# Autodesk Inventor assembly: MECANISMO DE COMPACTADO
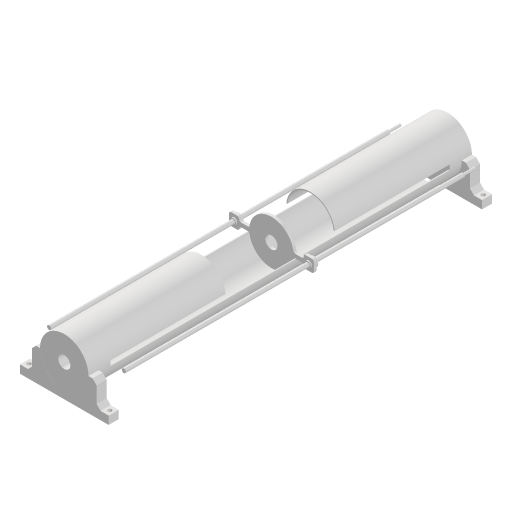
[picture p0: Inventor's stored thumbnail of the model, 512x512]
Saved by Autodesk Inventor 2024 (Build 280153000, 153)
## iProperties
Created: 2024-05-26
Part Number: MECANISMO DE COMPACTADO
Document SubType Name: Assembly
Designer: Jhuliams
Author: Jhuliams
## Documents named in this file (6)
- C:\Users\Jhuliams\Documents\GitHub\RECICLADOR_MODELO_3D\MECANISMO DE COMPACTADO\MECANISMO DE COMPACTADO.iam
- C:\Users\Jhuliams\Documents\GitHub\RECICLADOR_MODELO_3D\MECANISMO DE COMPACTADO\GUIA_DE_OBJETO.ipt
- C:\Users\Jhuliams\Documents\GitHub\RECICLADOR_MODELO_3D\MECANISMO DE COMPACTADO\TAPA QUE DESPLAZA CON TORNILLOS.ipt
- C:\Users\Jhuliams\Documents\GitHub\RECICLADOR_MODELO_3D\MECANISMO DE COMPACTADO\TUERCA DE HUSILLO.ipt
- C:\Users\Jhuliams\Documents\GitHub\RECICLADOR_MODELO_3D\MECANISMO DE COMPACTADO\TORNILLO DEPOTENCIA.ipt
- C:\Users\Jhuliams\Documents\GitHub\RECICLADOR_MODELO_3D\MECANISMO DE COMPACTADO\SOPORTE DE GUIA.ipt
## Components (8 placed, 5 different names)
1. GUIA_DE_OBJETO:1 — Mate:1, Mate:9, Mate:10, Mate:11, Mate:12, Mate:13, Flush:1, Flush:2
2. TAPA QUE DESPLAZA CON TORNILLOS:1 — Mate:1, Mate:3, Mate:4, Mate:5, Mate:6, Mate:11
3. TUERCA DE HUSILLO:1 — Mate:3, Mate:4, Mate:8
4. TUERCA DE HUSILLO:2 — Mate:5, Mate:6, Mate:7
5. TORNILLO DEPOTENCIA:1 — Mate:8, Mate:9
6. TORNILLO DEPOTENCIA:2 — Mate:7, Mate:10
7. SOPORTE DE GUIA:1 — Mate:12, Flush:1
8. SOPORTE DE GUIA:2 — Mate:13, Flush:2
## Relationships (14: Mate 12, Flush 2)
- Mate:1: GUIA_DE_OBJETO:1 ↔ TAPA QUE DESPLAZA CON TORNILLOS:1
- Mate:3: TAPA QUE DESPLAZA CON TORNILLOS:1 ↔ TUERCA DE HUSILLO:1
- Mate:4: TAPA QUE DESPLAZA CON TORNILLOS:1 ↔ TUERCA DE HUSILLO:1
- Mate:5: TAPA QUE DESPLAZA CON TORNILLOS:1 ↔ TUERCA DE HUSILLO:2
- Mate:6: TAPA QUE DESPLAZA CON TORNILLOS:1 ↔ TUERCA DE HUSILLO:2
- Mate:7: TUERCA DE HUSILLO:2 ↔ TORNILLO DEPOTENCIA:2
- Mate:8: TUERCA DE HUSILLO:1 ↔ TORNILLO DEPOTENCIA:1
- Mate:9: GUIA_DE_OBJETO:1 ↔ TORNILLO DEPOTENCIA:1
- Mate:10: GUIA_DE_OBJETO:1 ↔ TORNILLO DEPOTENCIA:2
- Mate:11 (1 mm): GUIA_DE_OBJETO:1 ↔ TAPA QUE DESPLAZA CON TORNILLOS:1
- Mate:12: GUIA_DE_OBJETO:1 ↔ SOPORTE DE GUIA:1
- Mate:13: GUIA_DE_OBJETO:1 ↔ SOPORTE DE GUIA:2
- Flush:1: GUIA_DE_OBJETO:1 ↔ SOPORTE DE GUIA:1
- Flush:2: GUIA_DE_OBJETO:1 ↔ SOPORTE DE GUIA:2
